# Autodesk Inventor assembly: backerBoardConnector
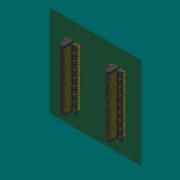
[picture p0: Inventor's stored thumbnail of the model, 180x180]
Saved by Autodesk Inventor 2016 (Build 200138000, 138)
## iProperties
Created: 2016-06-07
Part Number: backerBoardConnector
Document SubType Name: Assembly
Designer: sawaiz
Author: sawaiz
## Documents named in this file (3)
- C:\Users\sawaiz\oneDrive\projects\modularRICH\dependency\13361-30xxAE-08\backerBoardConnector.iam
- C:\Users\sawaiz\oneDrive\projects\modularRICH\dependency\13361-30xxAE-08\backerConnectorMount.ipt
- C:\Users\sawaiz\oneDrive\projects\modularRICH\dependency\13361-30xxAE-08\ST4-40-1.00-L-D-P-TR\ST4-40-1_00-L-D-P-TR.iam
## Components (3 placed, 2 different names)
1. backerConnectorMount:1 — Mate:1, Angle:1, Flush:1, Flush:2
2. ST4-40-1_00-L-D-P-TR:1 [sub-assembly] — Mate:1, Angle:1, Flush:1, Flush:2
3. ST4-40-1_00-L-D-P-TR:2 [sub-assembly]
## Component patterns: (2 elements, first: ST4-40-1_00-L-D-P-TR:1)
## Relationships (4: Flush 2, Mate 1, Angle 1)
- Mate:1: backerConnectorMount:1 ↔ ST4-40-1_00-L-D-P-TR:1
- Angle:1 (0 deg): backerConnectorMount:1 ↔ ST4-40-1_00-L-D-P-TR:1
- Flush:1 (0.025 mm): backerConnectorMount:1 ↔ ST4-40-1_00-L-D-P-TR:1
- Flush:2: backerConnectorMount:1 ↔ ST4-40-1_00-L-D-P-TR:1
